# Autodesk Inventor assembly: plataforma inteira20
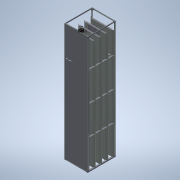
[picture p0: Inventor's stored thumbnail of the model, 180x180]
Saved by Autodesk Inventor 2020 (Build 240168000, 168)
## iProperties
Created: 2016-07-01
Part Number: plataforma inteira20
Document SubType Name: Assembly
Designer: New user
Mass: 4.89928e+06 g
Surface Area: 5.41775e+06 cm^2
Volume: 780204 cm^3
Density: 6.27948 g/cm^3
Author: New user
## Documents named in this file (8)
- C:\desk\Proj\inventor\plataforma inteira20.iam
- C:\desk\Proj\inventor\plataforma.iam
- C:\desk\Proj\inventor\suporte longitudinal.ipt
- C:\desk\Proj\inventor\plataformafrt.iam
- C:\desk\Proj\inventor\corners40hicube.iam
- C:\desk\Proj\inventor\suporte transversal.ipt
- C:\desk\Proj\inventor\suporte alto.ipt
- C:\desk\Proj\inventor\drone1.iam
## Components (18 placed, 7 different names)
1. plataforma:2 [sub-assembly] — Flush:2, Flush:6, Mate:3, Flush:7, Flush:8
2. plataforma:3 [sub-assembly] — Flush:1, Flush:2, Flush:5, Flush:6, Mate:1, Mate:3
3. plataforma:4 [sub-assembly] — Flush:1, Flush:5, Mate:1
4. suporte longitudinal:1 — Flush:18, Flush:19, Mate:14
5. suporte longitudinal:2 — Mate:11, Flush:20, Mate:16
6. plataformafrt:1 [sub-assembly] — Flush:7, Flush:8, Flush:9, Mate:11, Mate:22, Flush:33
7. corners40hicube:1 [sub-assembly] — Flush:9, Mate:7, Mate:8, Mate:9, Mate:10, Flush:10, Mate:12, Mate:13, Flush:12, Flush:13, Flush:14, Flush:15, Flush:16, Flush:17, Flush:18, Flush:19, Mate:14, Mate:15, Flush:20, Mate:16, Flush:21, Flush:22, Mate:17, Flush:23, Flush:24, Mate:18, Flush:25, Flush:26, Flush:27, Flush:28, Mate:19, Flush:29, Flush:30, Mate:20, Flush:31, Flush:32, Mate:21
8. suporte longitudinal:3 — Mate:10, Flush:10, Flush:11, Flush:14, Mate:22, Flush:33
9. suporte longitudinal:4 — Mate:12, Flush:11, Flush:17
10. suporte transversal:1 — Mate:7, Mate:13, Flush:15, Flush:16
11. suporte transversal:2 — Mate:8, Flush:12, Flush:13
12. suporte transversal:3 — Mate:9, Mate:15, Flush:21, Flush:22
13. suporte transversal:4 — Mate:17, Flush:23, Flush:24
14. suporte alto:1 — Mate:18, Flush:25, Flush:26
15. suporte alto:2 — Flush:27, Flush:28, Mate:19
16. suporte alto:3 — Flush:29, Flush:30, Mate:20
17. suporte alto:4 — Flush:31, Flush:32, Mate:21
18. drone1:2 [sub-assembly]
## Relationships (50: Flush 31, Mate 19)
- Flush:1: plataforma:3 ↔ plataforma:4
- Flush:2: plataforma:2 ↔ plataforma:3
- Flush:5: plataforma:3 ↔ plataforma:4
- Flush:6: plataforma:2 ↔ plataforma:3
- Mate:1: plataforma:3 ↔ plataforma:4
- Mate:3: plataforma:2 ↔ plataforma:3
- Flush:7: plataforma:2 ↔ plataformafrt:1
- Flush:8: plataforma:2 ↔ plataformafrt:1
- Flush:9: plataformafrt:1 ↔ corners40hicube:1
- Mate:7: corners40hicube:1 ↔ suporte transversal:1
- Mate:8: corners40hicube:1 ↔ suporte transversal:2
- Mate:9: corners40hicube:1 ↔ suporte transversal:3
- Mate:10: corners40hicube:1 ↔ suporte longitudinal:3
- Flush:10 (10 mm): corners40hicube:1 ↔ suporte longitudinal:3
- Mate:11: suporte longitudinal:2 ↔ plataformafrt:1
- Mate:12: corners40hicube:1 ↔ suporte longitudinal:4
- Flush:11: suporte longitudinal:3 ↔ suporte longitudinal:4
- Mate:13: corners40hicube:1 ↔ suporte transversal:1
- Flush:12: corners40hicube:1 ↔ suporte transversal:2
- Flush:13 (-10 mm): corners40hicube:1 ↔ suporte transversal:2
- Flush:14: corners40hicube:1 ↔ suporte longitudinal:3
- Flush:15 (-10 mm): corners40hicube:1 ↔ suporte transversal:1
- Flush:16: corners40hicube:1 ↔ suporte transversal:1
- Flush:17: corners40hicube:1 ↔ suporte longitudinal:4
- Flush:18 (-10 mm): suporte longitudinal:1 ↔ corners40hicube:1
- Flush:19 (-10 mm): suporte longitudinal:1 ↔ corners40hicube:1
- Mate:14: suporte longitudinal:1 ↔ corners40hicube:1
- Mate:15: corners40hicube:1 ↔ suporte transversal:3
- Flush:20: suporte longitudinal:2 ↔ corners40hicube:1
- Mate:16: suporte longitudinal:2 ↔ corners40hicube:1
- Flush:21: corners40hicube:1 ↔ suporte transversal:3
- Flush:22: corners40hicube:1 ↔ suporte transversal:3
- Mate:17: corners40hicube:1 ↔ suporte transversal:4
- Flush:23 (-10 mm): corners40hicube:1 ↔ suporte transversal:4
- Flush:24 (-10 mm): corners40hicube:1 ↔ suporte transversal:4
- Mate:18: corners40hicube:1 ↔ suporte alto:1
- Flush:25: corners40hicube:1 ↔ suporte alto:1
- Flush:26: corners40hicube:1 ↔ suporte alto:1
- Flush:27: corners40hicube:1 ↔ suporte alto:2
- Flush:28: corners40hicube:1 ↔ suporte alto:2
- Mate:19: corners40hicube:1 ↔ suporte alto:2
- Flush:29: corners40hicube:1 ↔ suporte alto:3
- Flush:30: corners40hicube:1 ↔ suporte alto:3
- Mate:20: corners40hicube:1 ↔ suporte alto:3
- Flush:31 (-10 mm): corners40hicube:1 ↔ suporte alto:4
- Flush:32 (-10 mm): corners40hicube:1 ↔ suporte alto:4
- Mate:21: corners40hicube:1 ↔ suporte alto:4
- Mate:22: plataformafrt:1 ↔ suporte longitudinal:3
- Flush:33: plataformafrt:1 ↔ suporte longitudinal:3
- [Mate] (10 mm): plataformafrt:1 ↔ drone1:2
